# Autodesk Inventor assembly: motor mount plate
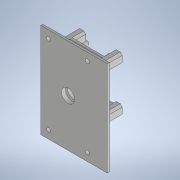
[picture p0: Inventor's stored thumbnail of the model, 180x180]
Saved by Autodesk Inventor 2022 (Build 260153000, 153)
## iProperties
Created: 2021-11-30
Part Number: motor mount plate
Document SubType Name: Assembly
Designer: a-dubs
Author: a-dubs
## Documents named in this file (3)
- W:\My Drive\Coding and Projects\smart home\smart-deadbolt\3D Modelling\motor mount plate.iam
- W:\My Drive\Coding and Projects\smart home\smart-deadbolt\3D Modelling\motor mount layer.ipt
- W:\My Drive\Coding and Projects\smart home\smart-deadbolt\3D Modelling\motor holder under.ipt
## Components (2 placed, 2 different names)
1. motor mount layer:1 — Mate:1, Mate:4
2. motor holder under:1 — Mate:1, Mate:4
## Relationships (2: Mate 2)
- Mate:1: motor mount layer:1 ↔ motor holder under:1
- Mate:4: motor mount layer:1 ↔ motor holder under:1
